# Autodesk Inventor assembly: jumper_completo
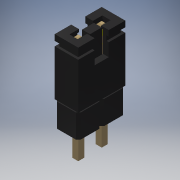
[picture p0: Inventor's stored thumbnail of the model, 180x180]
Saved by Autodesk Inventor 2019 (Build 230136000, 136)
## iProperties
Created: 2019-03-13
Part Number: jumper_completo
Material: Generico
Document SubType Name: Assembly
Designer: Thartarus
Author: Thartarus
## Documents named in this file (3)
- D:\KiCad eda\progetti kicad\SAE_Fenice\BMS_HV\CellsBoard\v2.1.1\modules\packages3d\jumper_completo.iam
- D:\KiCad eda\progetti kicad\SAE_Fenice\BMS_HV\CellsBoard\v2.1.1\modules\packages3d\jumper.ipt
- D:\KiCad eda\progetti kicad\SAE_Fenice\BMS_HV\CellsBoard\v2.1.1\modules\packages3d\SNT-100-BK-T\SNT-100-BK-T.ipt
## Components (2 placed, 2 different names)
1. jumper:1 — Coincidente:1, Coincidente:2, Coincidente:3, Allineato:1, Allineato:2, Coincidente:4
2. SNT-100-BK-T:1 — Allineato:1, Allineato:2, Coincidente:4
## Relationships (6: Mate 4, Flush 2)
- Coincidente:1 [Mate]: jumper:1
- Coincidente:2 [Mate] (-0.32 mm): jumper:1
- Coincidente:3 [Mate] (-0.32 mm): jumper:1
- Allineato:1 [Flush]: jumper:1 ↔ SNT-100-BK-T:1
- Allineato:2 [Flush]: jumper:1 ↔ SNT-100-BK-T:1
- Coincidente:4 [Mate] (0.1 mm): jumper:1 ↔ SNT-100-BK-T:1
